# Autodesk Inventor assembly: Assembly1
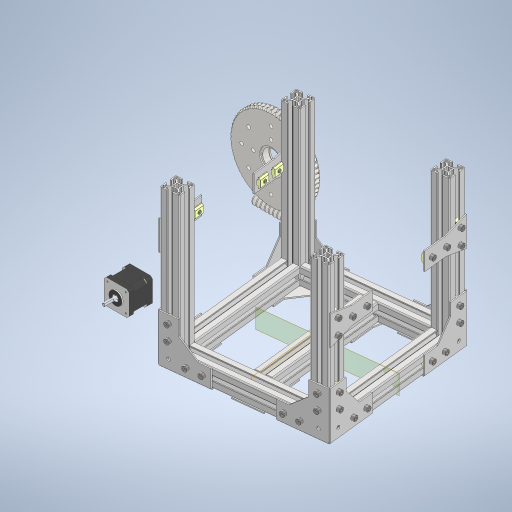
[picture p0: Inventor's stored thumbnail of the model, 512x512]
Saved by Autodesk Inventor 2024 (Build 280153000, 153)
## iProperties
Created: 2025-12-08
Part Number: Assembly1
Document SubType Name: Assembly
Designer: schar
Author: schar
## Documents named in this file (14)
- C:\Users\schar\Desktop\projectBlueprint\AMSTS\hardware\Assembly1.iam
- C:\Users\schar\Desktop\projectBlueprint\AMSTS\hardware\3030_200.ipt
- C:\Users\schar\Desktop\projectBlueprint\AMSTS\hardware\Connect2x3030_m6.ipt
- C:\Users\schar\Desktop\projectBlueprint\AMSTS\hardware\3030_tnut_m6.ipt
- C:\Users\schar\Documents\Inventor\Content Center Files\R2024\en-US\AS 1420\AS 1420 - 1973 - M5 x 10.ipt
- C:\Users\schar\Desktop\projectBlueprint\AMSTS\hardware\3030_260.ipt
- C:\Users\schar\Desktop\projectBlueprint\AMSTS\hardware\3030_connector_assembled.iam
- C:\Users\schar\Desktop\projectBlueprint\AMSTS\hardware\3030_connector_assembled_MIR.iam
- C:\Users\schar\Desktop\projectBlueprint\AMSTS\hardware\3030_connector_assembled_MIR1.iam
- C:\Users\schar\Desktop\projectBlueprint\AMSTS\hardware\3030_connector_assembled_MIR_MIR.iam
- C:\Users\schar\Desktop\projectBlueprint\AMSTS\hardware\Assembly1\Design Accelerator\Worm Gears3.iam
- C:\Users\schar\Desktop\projectBlueprint\AMSTS\hardware\3030_T_connector_assembled.iam
- C:\Users\schar\Desktop\projectBlueprint\AMSTS\hardware\3030_T_connector_assembled_MIR1.iam
- C:\Users\schar\Desktop\projectBlueprint\AMSTS\hardware\NEMA 17 - MS17HD2.iam
## Components (61 placed, 13 different names)
1. Worm Gears:2 [sub-assembly]
2. 3030_T_connector_assembled:1 [sub-assembly] — Mate:43, Flush:17
3. 3030_T_connector_assembled:2 [sub-assembly] — Mate:42, Flush:16
4. 3030_T_connector_assembled_MIR1:1 [sub-assembly] — Mate:50, Flush:21
5. 3030_T_connector_assembled_MIR1:2 [sub-assembly] — Mate:49, Flush:20
6. NEMA 17 - MS17HD2:1 [sub-assembly]
7. 3030_T_connector_assembled:3 [sub-assembly] — Mate:45, Flush:18, Mate:47, Flush:19
8. 3030_200:5 — Mate:47, Mate:48, Flush:19, Mate:52, Flush:22
9. 3030_T_connector_assembled:4 [sub-assembly] — Mate:53, Flush:22, Flush:23
10. 3030_200:1 — Mate:1, Mate:2, Flush:1, Flush:2, Mate:4, Flush:5, Flush:6, Symmetry:1, Mate:30, Mate:45, Flush:18, Mate:48
11. 3030_200:2 — Mate:3, Flush:3, Flush:4, Mate:6, Flush:9, Flush:10, Symmetry:2
12. Connect2x3030_m6:1 — Mate:1, Mate:2, Flush:1, Flush:2, Mate:3, Flush:3, Flush:4, Rigid:1, Rotational:5, Rotational:6, Rotational:7, Insert:11, Insert:12, Insert:14, Insert:15, Mate:19, Mate:20, Mate:21, Mate:36, Mate:37
13. Connect2x3030_m6:2 — Mate:4, Flush:5, Flush:6, Mate:5, Flush:7, Flush:8, Rotational:1, Rotational:2, Rotational:3, Rotational:4, Insert:6, Insert:7, Insert:9, Insert:10, Mate:10, Mate:11, Mate:12, Mate:32, Mate:33
14. Connect2x3030_m6:3 — Mate:8, Flush:11, Flush:12, Rotational:12, Rotational:13, Rotational:14, Rotational:15, Insert:1, Insert:2, Insert:4, Insert:5, Mate:13, Mate:14, Mate:15, Mate:40, Mate:41
15. Connect2x3030_m6:4 — Mate:6, Flush:9, Flush:10, Mate:7, Flush:13, Mate:9, Flush:14, Rotational:8, Rotational:9, Rotational:10, Rotational:11, Insert:16, Insert:17, Insert:18, Insert:20, Mate:16, Mate:17, Mate:18, Mate:23, Flush:15, Mate:25
16. 3030_200:3 — Mate:5, Flush:7, Flush:8, Mate:8, Flush:11, Flush:12, Symmetry:2, Mate:52
17. 3030_200:4 — Flush:13, Mate:9, Flush:14, Symmetry:1, Mate:53, Flush:23
18. 3030_connector_assembled:1 [sub-assembly] — Mate:24, Mate:25, Mate:26
19. 3030_connector_assembled:2 [sub-assembly] — Mate:22, Mate:23, Flush:15, Mate:26
20. 3030_connector_assembled_MIR:1 [sub-assembly] — Mate:27, Mate:39, Mate:40
21. 3030_connector_assembled_MIR:2 [sub-assembly] — Mate:27, Mate:38, Mate:41
22. 3030_connector_assembled_MIR1:1 [sub-assembly] — Mate:28, Mate:34, Mate:37
23. 3030_connector_assembled_MIR1:2 [sub-assembly] — Mate:28, Mate:35, Mate:36
24. 3030_connector_assembled_MIR_MIR:1 [sub-assembly] — Mate:29, Mate:30, Mate:33
25. 3030_connector_assembled_MIR_MIR:2 [sub-assembly] — Mate:29, Mate:31, Mate:32
26. 3030_260:1 — Mate:10, Mate:11, Mate:12, Mate:31, Mate:49, Flush:20
27. 3030_260:2 — Mate:13, Mate:14, Mate:15, Mate:38, Mate:39, Mate:42, Flush:16
28. 3030_260:3 — Mate:16, Mate:17, Mate:18, Mate:22, Mate:24, Mate:43, Flush:17
29. 3030_260:4 — Mate:19, Mate:20, Mate:21, Mate:34, Mate:35, Mate:50, Flush:21
30. 3030_tnut_m6:1 — Rotational:12
31. 3030_tnut_m6:2 — Rotational:11
32. 3030_tnut_m6:3 — Rigid:1
33. 3030_tnut_m6:4 — Rotational:1
34. 3030_tnut_m6:5 — Rotational:13
35. 3030_tnut_m6:6 — Rotational:10
36. 3030_tnut_m6:7 — Rotational:5
37. 3030_tnut_m6:8 — Rotational:2
38. 3030_tnut_m6:9 — Rotational:15
39. 3030_tnut_m6:10 — Rotational:8
40. 3030_tnut_m6:11 — Rotational:6
41. 3030_tnut_m6:12 — Rotational:4
42. 3030_tnut_m6:13 — Rotational:14
43. 3030_tnut_m6:14 — Rotational:9
44. 3030_tnut_m6:15 — Rotational:7
45. 3030_tnut_m6:16 — Rotational:3
46. AS 1420 - Metric M5 x 10:1 — Insert:1
47. AS 1420 - Metric M5 x 10:2 — Insert:2
48. AS 1420 - Metric M5 x 10:4 — Insert:4
49. AS 1420 - Metric M5 x 10:5 — Insert:5
50. AS 1420 - Metric M5 x 10:6 — Insert:6
51. AS 1420 - Metric M5 x 10:7 — Insert:7
52. AS 1420 - Metric M5 x 10:9 — Insert:9
53. AS 1420 - Metric M5 x 10:10 — Insert:10
54. AS 1420 - Metric M5 x 10:11 — Insert:11
55. AS 1420 - Metric M5 x 10:12 — Insert:12
56. AS 1420 - Metric M5 x 10:14 — Insert:14
57. AS 1420 - Metric M5 x 10:15 — Insert:15
58. AS 1420 - Metric M5 x 10:16 — Insert:16
59. AS 1420 - Metric M5 x 10:17 — Insert:17
60. AS 1420 - Metric M5 x 10:18 — Insert:18
61. AS 1420 - Metric M5 x 10:20 — Insert:20
## Relationships (107: Mate 50, Flush 23, Insert 16, RevoluteJoint 15, Symmetry 2, WeldJoint 1)
- Mate:1: 3030_200:1 ↔ Connect2x3030_m6:1
- Mate:2: 3030_200:1 ↔ Connect2x3030_m6:1
- Flush:1: 3030_200:1 ↔ Connect2x3030_m6:1
- Flush:2 (30 mm): 3030_200:1 ↔ Connect2x3030_m6:1
- Mate:3: 3030_200:2 ↔ Connect2x3030_m6:1
- Flush:3 (30 mm): 3030_200:2 ↔ Connect2x3030_m6:1
- Flush:4: 3030_200:2 ↔ Connect2x3030_m6:1
- Mate:4: 3030_200:1 ↔ Connect2x3030_m6:2
- Flush:5 (-30 mm): 3030_200:1 ↔ Connect2x3030_m6:2
- Flush:6: 3030_200:1 ↔ Connect2x3030_m6:2
- Mate:5: Connect2x3030_m6:2 ↔ 3030_200:3
- Flush:7 (30 mm): Connect2x3030_m6:2 ↔ 3030_200:3
- Flush:8: Connect2x3030_m6:2 ↔ 3030_200:3
- Mate:6: 3030_200:2 ↔ Connect2x3030_m6:4
- Flush:9 (-30 mm): 3030_200:2 ↔ Connect2x3030_m6:4
- Flush:10: 3030_200:2 ↔ Connect2x3030_m6:4
- Mate:7: Connect2x3030_m6:4
- Mate:8: Connect2x3030_m6:3 ↔ 3030_200:3
- Flush:11 (-30 mm): Connect2x3030_m6:3 ↔ 3030_200:3
- Flush:12: Connect2x3030_m6:3 ↔ 3030_200:3
- Flush:13: Connect2x3030_m6:4 ↔ 3030_200:4
- Mate:9: Connect2x3030_m6:4 ↔ 3030_200:4
- Flush:14 (-30 mm): Connect2x3030_m6:4 ↔ 3030_200:4
- Rotational:1 [RevoluteJoint] (-0.357 mm): Connect2x3030_m6:2 ↔ 3030_tnut_m6:4
- Rotational:2 [RevoluteJoint] (-0.357 mm): Connect2x3030_m6:2 ↔ 3030_tnut_m6:8
- Rotational:3 [RevoluteJoint] (-0.357 mm): Connect2x3030_m6:2 ↔ 3030_tnut_m6:16
- Rotational:4 [RevoluteJoint] (-0.357 mm): Connect2x3030_m6:2 ↔ 3030_tnut_m6:12
- Rigid:1 [WeldJoint] (-0.357 mm): Connect2x3030_m6:1 ↔ 3030_tnut_m6:3
- Rotational:5 [RevoluteJoint] (-0.357 mm): Connect2x3030_m6:1 ↔ 3030_tnut_m6:7
- Rotational:6 [RevoluteJoint] (-0.357 mm): Connect2x3030_m6:1 ↔ 3030_tnut_m6:11
- Rotational:7 [RevoluteJoint] (-0.357 mm): Connect2x3030_m6:1 ↔ 3030_tnut_m6:15
- Rotational:8 [RevoluteJoint] (-0.357 mm): Connect2x3030_m6:4 ↔ 3030_tnut_m6:10
- Rotational:9 [RevoluteJoint] (-0.357 mm): Connect2x3030_m6:4 ↔ 3030_tnut_m6:14
- Rotational:10 [RevoluteJoint] (-0.357 mm): Connect2x3030_m6:4 ↔ 3030_tnut_m6:6
- Rotational:11 [RevoluteJoint] (-0.357 mm): Connect2x3030_m6:4 ↔ 3030_tnut_m6:2
- Rotational:12 [RevoluteJoint] (-0.357 mm): Connect2x3030_m6:3 ↔ 3030_tnut_m6:1
- Rotational:13 [RevoluteJoint]: Connect2x3030_m6:3 ↔ 3030_tnut_m6:5
- Rotational:14 [RevoluteJoint] (-0.357 mm): Connect2x3030_m6:3 ↔ 3030_tnut_m6:13
- Rotational:15 [RevoluteJoint] (-0.357 mm): Connect2x3030_m6:3 ↔ 3030_tnut_m6:9
- Insert:1: Connect2x3030_m6:3 ↔ AS 1420 - Metric M5 x 10:1
- Insert:2: Connect2x3030_m6:3 ↔ AS 1420 - Metric M5 x 10:2
- Insert:4: Connect2x3030_m6:3 ↔ AS 1420 - Metric M5 x 10:4
- Insert:5: Connect2x3030_m6:3 ↔ AS 1420 - Metric M5 x 10:5
- Insert:6: Connect2x3030_m6:2 ↔ AS 1420 - Metric M5 x 10:6
- Insert:7: Connect2x3030_m6:2 ↔ AS 1420 - Metric M5 x 10:7
- Insert:9: Connect2x3030_m6:2 ↔ AS 1420 - Metric M5 x 10:9
- Insert:10: Connect2x3030_m6:2 ↔ AS 1420 - Metric M5 x 10:10
- Insert:11: Connect2x3030_m6:1 ↔ AS 1420 - Metric M5 x 10:11
- Insert:12: Connect2x3030_m6:1 ↔ AS 1420 - Metric M5 x 10:12
- Insert:14: Connect2x3030_m6:1 ↔ AS 1420 - Metric M5 x 10:14
- Insert:15: Connect2x3030_m6:1 ↔ AS 1420 - Metric M5 x 10:15
- Insert:16: Connect2x3030_m6:4 ↔ AS 1420 - Metric M5 x 10:16
- Insert:17: Connect2x3030_m6:4 ↔ AS 1420 - Metric M5 x 10:17
- Insert:18: Connect2x3030_m6:4 ↔ AS 1420 - Metric M5 x 10:18
- Insert:20: Connect2x3030_m6:4 ↔ AS 1420 - Metric M5 x 10:20
- Mate:10: Connect2x3030_m6:2 ↔ 3030_260:1
- Mate:11: Connect2x3030_m6:2 ↔ 3030_260:1
- Mate:12: Connect2x3030_m6:2 ↔ 3030_260:1
- Mate:13: Connect2x3030_m6:3 ↔ 3030_260:2
- Mate:14: Connect2x3030_m6:3 ↔ 3030_260:2
- Mate:15: Connect2x3030_m6:3 ↔ 3030_260:2
- Mate:16: Connect2x3030_m6:4 ↔ 3030_260:3
- Mate:17: Connect2x3030_m6:4 ↔ 3030_260:3
- Mate:18: Connect2x3030_m6:4 ↔ 3030_260:3
- Mate:19: Connect2x3030_m6:1 ↔ 3030_260:4
- Mate:20: Connect2x3030_m6:1 ↔ 3030_260:4
- Mate:21: Connect2x3030_m6:1 ↔ 3030_260:4
- Symmetry:1: 3030_200:1 ↔ 3030_200:4
- Mate:22: 3030_connector_assembled:2 ↔ 3030_260:3
- Mate:23: Connect2x3030_m6:4 ↔ 3030_connector_assembled:2
- Flush:15: Connect2x3030_m6:4 ↔ 3030_connector_assembled:2
- Mate:24: 3030_connector_assembled:1 ↔ 3030_260:3
- Mate:25: Connect2x3030_m6:4 ↔ 3030_connector_assembled:1
- Mate:26: 3030_connector_assembled:1 ↔ 3030_connector_assembled:2
- Symmetry:2: 3030_200:2 ↔ 3030_200:3
- Mate:27: 3030_connector_assembled_MIR:1 ↔ 3030_connector_assembled_MIR:2
- Mate:28: 3030_connector_assembled_MIR1:1 ↔ 3030_connector_assembled_MIR1:2
- Mate:29: 3030_connector_assembled_MIR_MIR:1 ↔ 3030_connector_assembled_MIR_MIR:2
- Mate:30: 3030_200:1 ↔ 3030_connector_assembled_MIR_MIR:1
- Mate:31: 3030_connector_assembled_MIR_MIR:2 ↔ 3030_260:1
- Mate:32: Connect2x3030_m6:2 ↔ 3030_connector_assembled_MIR_MIR:2
- Mate:33: Connect2x3030_m6:2 ↔ 3030_connector_assembled_MIR_MIR:1
- Mate:34: 3030_connector_assembled_MIR1:1 ↔ 3030_260:4
- Mate:35: 3030_connector_assembled_MIR1:2 ↔ 3030_260:4
- Mate:36: Connect2x3030_m6:1 ↔ 3030_connector_assembled_MIR1:2
- Mate:37: Connect2x3030_m6:1 ↔ 3030_connector_assembled_MIR1:1
- Mate:38: 3030_connector_assembled_MIR:2 ↔ 3030_260:2
- Mate:39: 3030_connector_assembled_MIR:1 ↔ 3030_260:2
- Mate:40: Connect2x3030_m6:3 ↔ 3030_connector_assembled_MIR:1
- Mate:41: Connect2x3030_m6:3 ↔ 3030_connector_assembled_MIR:2
- Mate:42: 3030_T_connector_assembled:2 ↔ 3030_260:2
- Flush:16: 3030_T_connector_assembled:2 ↔ 3030_260:2
- Mate:43: 3030_T_connector_assembled:1 ↔ 3030_260:3
- Flush:17: 3030_T_connector_assembled:1 ↔ 3030_260:3
- Mate:45: 3030_T_connector_assembled:3 ↔ 3030_200:1
- Flush:18: 3030_T_connector_assembled:3 ↔ 3030_200:1
- Mate:47: 3030_T_connector_assembled:3 ↔ 3030_200:5
- Mate:48: 3030_200:5 ↔ 3030_200:1
- Flush:19: 3030_T_connector_assembled:3 ↔ 3030_200:5
- Mate:49: 3030_T_connector_assembled_MIR1:2 ↔ 3030_260:1
- Flush:20: 3030_T_connector_assembled_MIR1:2 ↔ 3030_260:1
- Mate:50: 3030_T_connector_assembled_MIR1:1 ↔ 3030_260:4
- Flush:21: 3030_T_connector_assembled_MIR1:1 ↔ 3030_260:4
- Mate:52 (90 mm): 3030_200:5 ↔ 3030_200:3
- Mate:53: 3030_T_connector_assembled:4 ↔ 3030_200:4
- Flush:22: 3030_200:5 ↔ 3030_T_connector_assembled:4
- Flush:23: 3030_T_connector_assembled:4 ↔ 3030_200:4
